# Autodesk Inventor assembly: HipRight
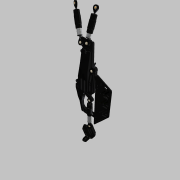
[picture p0: Inventor's stored thumbnail of the model, 180x180]
Saved by Autodesk Inventor 2015 (Build 190159000, 159)
## iProperties
Created: 2014-09-17
Part Number: HipRight
Document SubType Name: Assembly
Designer: Val
Mass: 921.173 g
Surface Area: 2138.12 cm^2
Volume: 469.881 cm^3
Density: 1.96044 g/cm^3
Author: Val
## Documents named in this file (9)
- E:\Exo\Moegìs\3D\HipRioht.iam
- G:\E<o\MoŤels\3D\HiѰFoTtgmConneãtorRi≧ht.ipt
- E:\Exo\M࡯dɥls\3D\HhpPopConŮ䁥c}ɯrRight.ipt
- E:\Exၯ\Models\3D\Ex4ernaѬ\BearingBody.ipt
- E:\Exo\ModEls\3D\BackPair1PistonBottomCap.ipt
- E:]Exo\Modelw\sD\BackPair1PၩstoŮShaft.ipt
- E:\Exo\Models\3D|BackPair1PistonTopCap.ipt
- E:\E䁸o\Models\3D\ShiŮConnectorSlider.ipt
- E:\Ex/\Models]3D\HipShock⃐lct聤Rioht.ipp
## Components (33 placed, 13 different names)
1. HipBottomConnectorRight:1 — Mate:3, Mate:4, Angle:1, Mate:9
2. HipPistonConnectorRight:1 — Mate:1, Mate:2, Mate:10, Mate:11
3. HipRight:1 — Mate:1, Mate:2, Mate:3, Mate:4, Angle:1, Mate:5, Mate:6, Angle:2, Mate:13, Mate:14, Mate:15, Mate:16, Mate:17, Mate:68, Mate:69
4. HipShockPlateRight:1 — Mate:7, Mate:8, Mate:9
5. HipTopConnectorRight:1 — Mate:5, Mate:6, Angle:2, Mate:7, Mate:8
6. BearingBall:1 — Mate:10, Mate:11, Mate:12
7. BearingBall:2 — Mate:68, Mate:69, Mate:70
8. BearingBall:3 — Mate:15, Mate:16, Mate:17, Mate:20
9. BearingBall:4 — Mate:13, Mate:14, Mate:19
10. BearingBody:1 — Mate:19, Mate:57
11. BearingBody:2 — Mate:20, Mate:58
12. BearingBody:4 — Mate:12, Mate:59
13. BackPair1PistonBody:2
14. BackPair1PistonBottomCap:2
15. BackPair1PistonShaft:2
16. BackPair1PistonTopCap:2 — Mate:57
17. BearingBody:6
18. BearingBall:6
19. BackPair1PistonBody:3
20. BackPair1PistonBottomCap:3
21. BackPair1PistonShaft:3
22. BackPair1PistonTopCap:3 — Mate:59, Mate:65
23. BackPair1PistonBody:4
24. BackPair1PistonBottomCap:4
25. BackPair1PistonShaft:4
26. BackPair1PistonTopCap:4 — Mate:58
27. BearingBody:8
28. BearingBall:8
29. ShinConnectorSliderLeft:1 — Mate:62, Mate:63, Mate:66, Mate:67, Angle:3
30. BearingBall:9 — Mate:62, Mate:63, Mate:64
31. BearingBody:9 — Mate:64, Mate:65
32. ShinConnectorRight:1 — Mate:66, Mate:67, Angle:3
33. BearingBody:10 — Mate:70
## Relationships (56: Mate 53, Angle 3)
- Mate:1: HipPistonConnectorRight:1 ↔ HipRight:1
- Mate:2: HipPistonConnectorRight:1 ↔ HipRight:1
- Mate:3: HipBottomConnectorRight:1 ↔ HipRight:1
- Mate:4: HipBottomConnectorRight:1 ↔ HipRight:1
- Angle:1 (0 deg): HipBottomConnectorRight:1 ↔ HipRight:1
- Mate:5: HipRight:1 ↔ HipTopConnectorRight:1
- Mate:6: HipRight:1 ↔ HipTopConnectorRight:1
- Angle:2 (0 deg): HipRight:1 ↔ HipTopConnectorRight:1
- Mate:7: HipShockPlateRight:1 ↔ HipTopConnectorRight:1
- Mate:8: HipShockPlateRight:1 ↔ HipTopConnectorRight:1
- Mate:9: HipBottomConnectorRight:1 ↔ HipShockPlateRight:1
- Mate:10: HipPistonConnectorRight:1 ↔ BearingBall:1
- Mate:11: HipPistonConnectorRight:1 ↔ BearingBall:1
- Mate:12: BearingBall:1 ↔ BearingBody:4
- Mate:13: HipRight:1 ↔ BearingBall:4
- Mate:14: HipRight:1 ↔ BearingBall:4
- Mate:15: HipRight:1 ↔ BearingBall:3
- Mate:16: HipRight:1 ↔ BearingBall:3
- Mate:17: HipRight:1 ↔ BearingBall:3
- Mate:19: BearingBall:4 ↔ BearingBody:1
- Mate:20: BearingBall:3 ↔ BearingBody:2
- [Mate]: BackPair1PistonBody:2 ↔ BackPair1PistonShaft:2
- [Mate]: BackPair1PistonBody:2 ↔ BackPair1PistonBottomCap:2
- [Mate]: BackPair1PistonBody:2 ↔ BackPair1PistonBottomCap:2
- [Mate]: BackPair1PistonShaft:2 ↔ BackPair1PistonTopCap:2
- [Mate]: BackPair1PistonShaft:2 ↔ BackPair1PistonTopCap:2
- [Mate]: BackPair1PistonShaft:2 ↔ BackPair1PistonTopCap:2
- [Mate]: BackPair1PistonBottomCap:2 ↔ BearingBody:6
- [Mate]: BearingBody:6 ↔ BearingBall:6
- [Mate]: BackPair1PistonBody:3 ↔ BackPair1PistonShaft:3
- [Mate]: BackPair1PistonBody:3 ↔ BackPair1PistonBottomCap:3
- [Mate]: BackPair1PistonBody:3 ↔ BackPair1PistonBottomCap:3
- [Mate]: BackPair1PistonShaft:3 ↔ BackPair1PistonTopCap:3
- [Mate]: BackPair1PistonShaft:3 ↔ BackPair1PistonTopCap:3
- [Mate]: BackPair1PistonShaft:3 ↔ BackPair1PistonTopCap:3
- [Mate]: BackPair1PistonBody:4 ↔ BackPair1PistonShaft:4
- [Mate]: BackPair1PistonBody:4 ↔ BackPair1PistonBottomCap:4
- [Mate]: BackPair1PistonBody:4 ↔ BackPair1PistonBottomCap:4
- [Mate]: BackPair1PistonShaft:4 ↔ BackPair1PistonTopCap:4
- [Mate]: BackPair1PistonShaft:4 ↔ BackPair1PistonTopCap:4
- [Mate]: BackPair1PistonShaft:4 ↔ BackPair1PistonTopCap:4
- [Mate]: BackPair1PistonBottomCap:4 ↔ BearingBody:8
- [Mate]: BearingBody:8 ↔ BearingBall:8
- Mate:57: BearingBody:1 ↔ BackPair1PistonTopCap:2
- Mate:58: BearingBody:2 ↔ BackPair1PistonTopCap:4
- Mate:59: BearingBody:4 ↔ BackPair1PistonTopCap:3
- Mate:62: ShinConnectorSliderLeft:1 ↔ BearingBall:9
- Mate:63: ShinConnectorSliderLeft:1 ↔ BearingBall:9
- Mate:64: BearingBall:9 ↔ BearingBody:9
- Mate:65: BackPair1PistonTopCap:3 ↔ BearingBody:9
- Mate:66: ShinConnectorSliderLeft:1 ↔ ShinConnectorRight:1
- Mate:67: ShinConnectorSliderLeft:1 ↔ ShinConnectorRight:1
- Angle:3 (0 deg): ShinConnectorSliderLeft:1 ↔ ShinConnectorRight:1
- Mate:68: HipRight:1 ↔ BearingBall:2
- Mate:69: HipRight:1 ↔ BearingBall:2
- Mate:70: BearingBall:2 ↔ BearingBody:10
## Named parameters: d31_d106 = 0 mm, d32_d83_d73 = 0 mm, d33_d84_d52 = 0 mm, d34_d85_d53 = 0 mm, d35_d86_d54 = 0 mm, d36_d87_d55 = 0 mm, d37_d88_d56 = 0 mm, d38_d89_d57 = 0 mm, d41_d84_d52 = 0 mm, d42_d85_d53 = 0 mm, d43_d86_d54 = 0 mm, d44_d87_d55 = 0 mm, d45_d88_d56 = 0 mm, d46_d89_d57 = 0 mm, d47_d106 = 0 mm, d48_d83_d73 = 0 mm, d49_d84_d52 = 0 mm, d50_d85_d53 = 0 mm, d51_d86_d54 = 0 mm, d52_d87_d55 = 0 mm, d53_d88_d56 = 0 mm, d54_d89_d57 = 0 mm
